# Autodesk Inventor assembly: V5SlapperTower
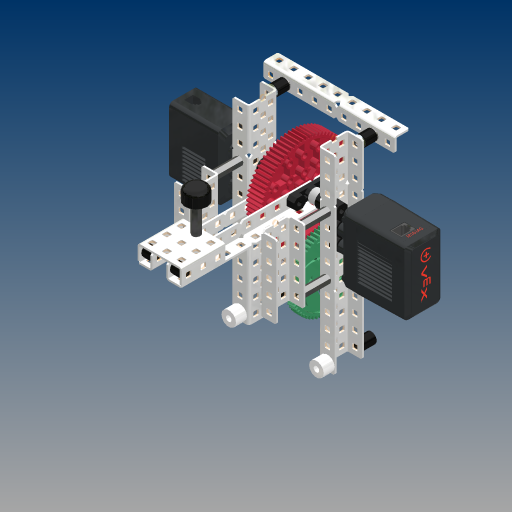
[picture p0: Inventor's stored thumbnail of the model, 512x512]
Saved by Autodesk Inventor 2023 (Build 270158000, 158)
## iProperties
Created: 2024-02-14
Part Number: V5SlapperTower
Document SubType Name: Assembly
Designer: eddie
Author: eddie
## Documents named in this file (26)
- C:\Users\eddie\Documents\81208X-Over-Under-CAD\V5\V5SlapperTower.iam
- C:\Users\eddie\Documents\81208X-Over-Under-CAD\VEX-CAD-Inventor-1.4.0\Structure\C Channel\Aluminum 1x2x1\Alu C 1x2x1x13.ipt
- C:\Users\eddie\Documents\81208X-Over-Under-CAD\VEX-CAD-Inventor-1.4.0\Motion\Spacers\Spacer Nylon .375 OD\NSpacer .375 OD x .500.ipt
- C:\Users\eddie\Documents\81208X-Over-Under-CAD\VEX-CAD-Inventor-1.4.0\Motion\Spacers\Spacer Nylon .375 OD.ipt
- C:\Users\eddie\Documents\81208X-Over-Under-CAD\VEX-CAD-Inventor-1.4.0\Structure\Hardware\Nut Keps.ipt
- C:\Users\eddie\Documents\81208X-Over-Under-CAD\VEX-CAD-Inventor-1.4.0\Motion\Spacers\Spacer Nylon .375 OD\NSpacer .375 OD x .375.ipt
- C:\Users\eddie\Documents\81208X-Over-Under-CAD\VEX-CAD-Inventor-1.4.0\Motion\Spacers\Washer Steel\SWasher .375 OD x .031250.ipt
- C:\Users\eddie\Documents\81208X-Over-Under-CAD\VEX-CAD-Inventor-1.4.0\Motion\Spacers\Washer Steel.ipt
- C:\Users\eddie\Documents\81208X-Over-Under-CAD\VEX-CAD-Inventor-1.4.0\Structure\Angle\Aluminum\1x1\Alu Angle 1x1x9.ipt
- C:\Users\eddie\Documents\81208X-Over-Under-CAD\VEX-CAD-Inventor-1.4.0\Structure\Standoff\Standoff 1.00.ipt
- C:\Users\eddie\Documents\81208X-Over-Under-CAD\VEX-CAD-Inventor-1.4.0\Structure\Standoff.ipt
- C:\Users\eddie\Documents\81208X-Over-Under-CAD\VEX-CAD-Inventor-1.4.0\Structure\C Channel\Aluminum 1x2x1\Alu C 1x2x1x5.ipt
- C:\Users\eddie\Documents\81208X-Over-Under-CAD\VEX-CAD-Inventor-1.4.0\Motion\Spacers\Spacer Nylon .500 OD\NSpacer Black .500 OD x .375.ipt
- C:\Users\eddie\Documents\81208X-Over-Under-CAD\VEX-CAD-Inventor-1.4.0\Motion\Spacers\Spacer Nylon .500 OD.ipt
- C:\Users\eddie\Documents\81208X-Over-Under-CAD\Custom-parts\Shaft Collar.ipt
- C:\Users\eddie\Documents\81208X-Over-Under-CAD\VEX-CAD-Inventor-1.4.0\Structure\Angle\Aluminum\1x1\Alu Angle 1x1x12.ipt
- C:\Users\eddie\Documents\81208X-Over-Under-CAD\VEX-CAD-Inventor-1.4.0\Motion\Shaft LS\Bearing Flat.ipt
- C:\Users\eddie\Documents\81208X-Over-Under-CAD\VEX-CAD-Inventor-1.4.0\Motion\Gears\HS Gear.iam
- C:\Users\eddie\Documents\81208X-Over-Under-CAD\VEX-CAD-Inventor-1.4.0\Structure\C Channel\Aluminum 1x3x1\Alu C 1x3x1x3.ipt
- C:\Users\eddie\Documents\81208X-Over-Under-CAD\VEX-CAD-Inventor-1.4.0\Structure\Hardware\Rubber Bumper Threaded.ipt
- C:\Users\eddie\Documents\81208X-Over-Under-CAD\VEX-CAD-Inventor-1.4.0\Motion\Gears\LS 60T Gear.ipt
- C:\Users\eddie\Documents\81208X-Over-Under-CAD\VEX-CAD-Inventor-1.4.0\Motion\Gears\HS Gear\HS 24T Gear, Square.iam
- C:\Users\eddie\Documents\81208X-Over-Under-CAD\VEX-CAD-Inventor-1.4.0\Motion\Gears\HS Gear\HS 72T Gear, Square.iam
- C:\Users\eddie\Documents\81208X-Over-Under-CAD\VEX-CAD-Inventor-1.4.0\Motion\Spacers\Spacer Nylon .500 OD\NSpacer White .500 OD x .375.ipt
- C:\Users\eddie\Documents\81208X-Over-Under-CAD\VEX-CAD-Inventor-1.4.0\Electronics\V5 Motor.ipt
- C:\Users\eddie\Documents\81208X-Over-Under-CAD\Custom-parts\5.5w_Motor.ipt
## Components (48 placed, 20 different names)
1. Alu C 1x2x1x13:1 — Insert:18, Insert:26, Insert:48, Insert:54, Insert:55, Insert:61, Insert:64
2. Alu C 1x2x1x13:2 — Insert:17, Insert:27, Insert:35, Insert:47, Insert:57, Insert:58, Insert:60, Insert:62
3. NSpacer Black .500 OD x .375:1 — Insert:18, Insert:20
4. NSpacer Black .500 OD x .375:2 — Insert:17, Insert:19
5. Shaft Collar:1 — Insert:19, Insert:23
6. Shaft Collar:2 — Insert:20, Insert:24
7. Alu Angle 1x1x12:1 — Insert:22, Insert:29, Insert:43
8. Alu Angle 1x1x12:2 — Insert:21, Insert:28
9. Bearing Flat:1 — Insert:22, Insert:23
10. Bearing Flat:2 — Insert:21, Insert:24
11. Alu C 1x3x1x3:1 — Insert:30, Insert:31
12. NSpacer .375 OD x .500:7 — Insert:27
13. NSpacer .375 OD x .500:8 — Insert:26
14. NSpacer .375 OD x .375:9 — Insert:29
15. NSpacer .375 OD x .375:10 — Insert:28, Insert:30
16. Standoff 1.00:5 — Insert:31, Insert:32
17. Rubber Bumper Threaded:1 — Insert:32
18. HS 24T Gear, Square:3 [sub-assembly] — Insert:42, Insert:44
19. NSpacer Black .500 OD x .375:4 — Insert:40, Insert:41
20. SWasher .375 OD x .031250:8 — Insert:39, Insert:40
21. SWasher .375 OD x .031250:9 — Insert:38, Insert:39
22. SWasher .375 OD x .031250:10 — Insert:35, Insert:36
23. LS 60T Gear:2 — Insert:37, Insert:38
24. SWasher .375 OD x .031250:13 — Insert:36, Insert:37
25. SWasher .375 OD x .031250:14 — Insert:41, Insert:42
26. HS 72T Gear, Square:4 [sub-assembly] — Insert:43
27. Shaft Collar:3 — Insert:44, Insert:45
28. NSpacer .375 OD x .500:11 — Insert:45, Insert:46
29. Shaft Collar:4 — Insert:46
30. Nut Keps:3 — Insert:48, Insert:50
31. Nut Keps:4 — Insert:47, Insert:49
32. NSpacer .375 OD x .375:12 — Insert:49, Insert:51
33. NSpacer .375 OD x .375:13 — Insert:50, Insert:52
34. SWasher .375 OD x .031250:15 — Insert:52, Insert:53
35. SWasher .375 OD x .031250:16 — Insert:51
36. Alu Angle 1x1x9:3 — Insert:53
37. Standoff 1.00:6 — Insert:54, Insert:56
38. Standoff 1.00:7 — Insert:55
39. Alu C 1x2x1x5:3 — Insert:56
40. Standoff 1.00:8 — Insert:57, Insert:59
41. Standoff 1.00:9 — Insert:58
42. Alu C 1x2x1x5:4 — Insert:59
43. NSpacer White .500 OD x .375:5 — Insert:60
44. NSpacer White .500 OD x .375:6 — Insert:61
45. V5 Motor:1 — Insert:63
46. Bearing Flat:3 — Insert:62, Insert:63
47. Bearing Flat:4 — Insert:64, Insert:65
48. 5.5w_Motor:1 — Insert:65
## Relationships (46: Insert 46)
- Insert:17: Alu C 1x2x1x13:2 ↔ NSpacer Black .500 OD x .375:2
- Insert:18: Alu C 1x2x1x13:1 ↔ NSpacer Black .500 OD x .375:1
- Insert:19: NSpacer Black .500 OD x .375:2 ↔ Shaft Collar:1
- Insert:20: NSpacer Black .500 OD x .375:1 ↔ Shaft Collar:2
- Insert:21: Alu Angle 1x1x12:2 ↔ Bearing Flat:2
- Insert:22: Alu Angle 1x1x12:1 ↔ Bearing Flat:1
- Insert:23: Shaft Collar:1 ↔ Bearing Flat:1
- Insert:24: Shaft Collar:2 ↔ Bearing Flat:2
- Insert:26: Alu C 1x2x1x13:1 ↔ NSpacer .375 OD x .500:8
- Insert:27: Alu C 1x2x1x13:2 ↔ NSpacer .375 OD x .500:7
- Insert:28: Alu Angle 1x1x12:2 ↔ NSpacer .375 OD x .375:10
- Insert:29: Alu Angle 1x1x12:1 ↔ NSpacer .375 OD x .375:9
- Insert:30: Alu C 1x3x1x3:1 ↔ NSpacer .375 OD x .375:10
- Insert:31: Alu C 1x3x1x3:1 ↔ Standoff 1.00:5
- Insert:32: Standoff 1.00:5 ↔ Rubber Bumper Threaded:1
- Insert:35: Alu C 1x2x1x13:2 ↔ SWasher .375 OD x .031250:10
- Insert:36: SWasher .375 OD x .031250:10 ↔ SWasher .375 OD x .031250:13
- Insert:37: LS 60T Gear:2 ↔ SWasher .375 OD x .031250:13
- Insert:38: SWasher .375 OD x .031250:9 ↔ LS 60T Gear:2
- Insert:39: SWasher .375 OD x .031250:8 ↔ SWasher .375 OD x .031250:9
- Insert:40: NSpacer Black .500 OD x .375:4 ↔ SWasher .375 OD x .031250:8
- Insert:41: NSpacer Black .500 OD x .375:4 ↔ SWasher .375 OD x .031250:14
- Insert:42: HS 24T Gear, Square:3 ↔ SWasher .375 OD x .031250:14
- Insert:43: Alu Angle 1x1x12:1 ↔ HS 72T Gear, Square:4
- Insert:44: HS 24T Gear, Square:3 ↔ Shaft Collar:3
- Insert:45: Shaft Collar:3 ↔ NSpacer .375 OD x .500:11
- Insert:46: NSpacer .375 OD x .500:11 ↔ Shaft Collar:4
- Insert:47: Alu C 1x2x1x13:2 ↔ Nut Keps:4
- Insert:48: Alu C 1x2x1x13:1 ↔ Nut Keps:3
- Insert:49: Nut Keps:4 ↔ NSpacer .375 OD x .375:12
- Insert:50: Nut Keps:3 ↔ NSpacer .375 OD x .375:13
- Insert:51: NSpacer .375 OD x .375:12 ↔ SWasher .375 OD x .031250:16
- Insert:52: NSpacer .375 OD x .375:13 ↔ SWasher .375 OD x .031250:15
- Insert:53: SWasher .375 OD x .031250:15 ↔ Alu Angle 1x1x9:3
- Insert:54: Alu C 1x2x1x13:1 ↔ Standoff 1.00:6
- Insert:55: Alu C 1x2x1x13:1 ↔ Standoff 1.00:7
- Insert:56: Standoff 1.00:6 ↔ Alu C 1x2x1x5:3
- Insert:57: Alu C 1x2x1x13:2 ↔ Standoff 1.00:8
- Insert:58: Alu C 1x2x1x13:2 ↔ Standoff 1.00:9
- Insert:59: Standoff 1.00:8 ↔ Alu C 1x2x1x5:4
- Insert:60: Alu C 1x2x1x13:2 ↔ NSpacer White .500 OD x .375:5
- Insert:61: Alu C 1x2x1x13:1 ↔ NSpacer White .500 OD x .375:6
- Insert:62: Alu C 1x2x1x13:2 ↔ Bearing Flat:3
- Insert:63: V5 Motor:1 ↔ Bearing Flat:3
- Insert:64: Alu C 1x2x1x13:1 ↔ Bearing Flat:4
- Insert:65: Bearing Flat:4 ↔ 5.5w_Motor:1
